# Autodesk Inventor assembly: First_Gear_Assembly
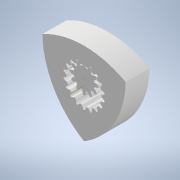
[picture p0: Inventor's stored thumbnail of the model, 180x180]
Saved by Autodesk Inventor 2021 (Build 250183000, 183)
## iProperties
Created: 2021-03-25
Part Number: First_Gear_Assembly
Document SubType Name: Assembly
Designer: lucia
Author: lucia
## Documents named in this file (3)
- E:\Documents\Inventor\Fixed Rotor Wankel Engine\Parts\First_Gear_Assembly.iam
- E:\Documents\Inventor\Fixed Rotor Wankel Engine\Parts\Rotor_Geared.ipt
- E:\Documents\Inventor\Fixed Rotor Wankel Engine\Parts\12_Tooth_Gear.ipt
## Components (2 placed, 2 different names)
1. Rotor_Geared:1 — Mate:1, Mate:3, Flush:1, Flush:2, Rotation:1
2. 12_Tooth_Gear:1 — Flush:2, Mate:4, Rotation:1
## Relationships (9: Mate 6, Flush 2, RelateRotation 1)
- Mate:1: Rotor_Geared:1
- Mate:2
- Mate:3: Rotor_Geared:1
- Flush:1: Rotor_Geared:1
- Flush:2: Rotor_Geared:1 ↔ 12_Tooth_Gear:1
- Mate:4: 12_Tooth_Gear:1
- Mate:5
- Mate:6 (13.208 mm)
- Rotation:1 [RelateRotation] (0.6667 ul): Rotor_Geared:1 ↔ 12_Tooth_Gear:1
